# Autodesk Inventor assembly: Canne final
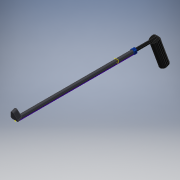
[picture p0: Inventor's stored thumbnail of the model, 180x180]
Saved by Autodesk Inventor 2018.1 (Build 221171000, 171)
## iProperties
Created: 2019-11-22
Part Number: Canne final
Material: Générique
Document SubType Name: Assembly
Designer: Tgremling1
Author: Tgremling1
## Documents named in this file (5)
- F:\EPI SIMU\Canne final.iam
- F:\EPI SIMU\Bas du manche.ipt
- F:\EPI SIMU\Goupille.ipt
- F:\EPI SIMU\Haut du manche.ipt
- F:\EPI SIMU\Vis.ipt
## Components (4 placed, 4 different names)
1. Bas du manche:1 — Affleurement:1, Affleurement:2, Affleurement:3, Placage:1, Affleurement:4
2. Goupille:1 — Affleurement:3, Placage:1, Affleurement:4, Logement:1
3. Haut du manche:1 — Affleurement:1, Affleurement:2
4. Vis:1 — Logement:1
## Relationships (6: Flush 4, Mate 1, Insert 1)
- Affleurement:1 [Flush] (3.01 mm): Bas du manche:1 ↔ Haut du manche:1
- Affleurement:2 [Flush] (3.01 mm): Bas du manche:1 ↔ Haut du manche:1
- Affleurement:3 [Flush] (-3 mm): Bas du manche:1 ↔ Goupille:1
- Placage:1 [Mate]: Bas du manche:1 ↔ Goupille:1
- Affleurement:4 [Flush]: Bas du manche:1 ↔ Goupille:1
- Logement:1 [Insert]: Goupille:1 ↔ Vis:1
